# Autodesk Inventor assembly: game assembly
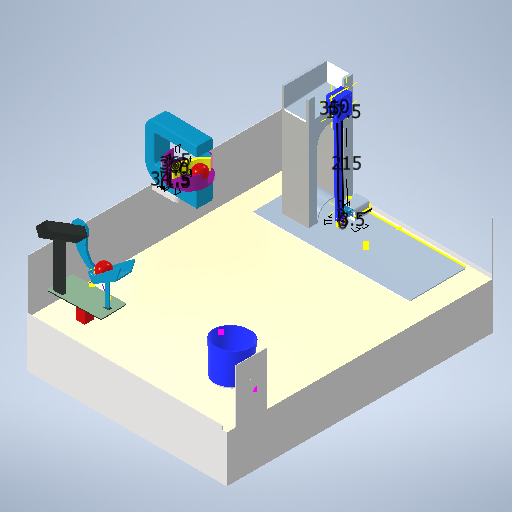
[picture p0: Inventor's stored thumbnail of the model, 512x512]
Saved by Autodesk Inventor 2025.4 (Build 294407000, 407)
## iProperties
Created: 2026-03-18
Part Number: game assembly
Document SubType Name: Assembly
Designer: youse
Author: youse
## Documents named in this file (6)
- D:\basics project\game assembly.iam
- D:\basics project\game base.ipt
- D:\basics project\Lifting Mechanism (2)\Lifting Mechanism\Lifting Mechanism.iam
- D:\basics project\shooting Mechanism - Copy.iam
- D:\basics project\السلة\CAD\Assembly1.iam
- D:\basics project\Basics of Mechatronics\Basics of Mechatronics\Assembly2.iam
## Components (5 placed, 5 different names)
1. game base:1 — Mate:1, Mate:2, Mate:3, Mate:4, Mate:5
2. Lifting Mechanism:1 [sub-assembly] — Mate:1
3. shooting Mechanism - Copy:1 [sub-assembly] — Mate:3, Mate:4
4. Assembly1:1 [sub-assembly] — Mate:5
5. Assembly2:1 [sub-assembly] — Mate:2
## Relationships (5: Mate 5)
- Mate:1: game base:1 ↔ Lifting Mechanism:1
- Mate:2: game base:1 ↔ Assembly2:1
- Mate:3: game base:1 ↔ shooting Mechanism - Copy:1
- Mate:4: game base:1 ↔ shooting Mechanism - Copy:1
- Mate:5: game base:1 ↔ Assembly1:1
## Named parameters: Finish1_Area = 362.6, Finish1_Thickness = 0.05 mm, Finish2_Area = 24, Finish2_Thickness = 0.05 mm, Finish3_Area = 47.9101, Finish3_Thickness = 0.05 mm, Finish4_Area = 10, Finish4_Thickness = 0.05 mm, Finish5_Area = 2668.21, Finish5_Thickness = 0.05 mm, Finish6_Area = 69.2254, Finish6_Thickness = 0.05 mm, Finish7_Area = 47.1689, Finish7_Thickness = 0.05 mm
note: some values were not read from the file. Shown as the stored number, unit unknown: "Finish1_Area", "Finish2_Area", "Finish3_Area", "Finish4_Area", "Finish5_Area", "Finish6_Area", "Finish7_Area".
